# Autodesk Inventor assembly: chess-set-one
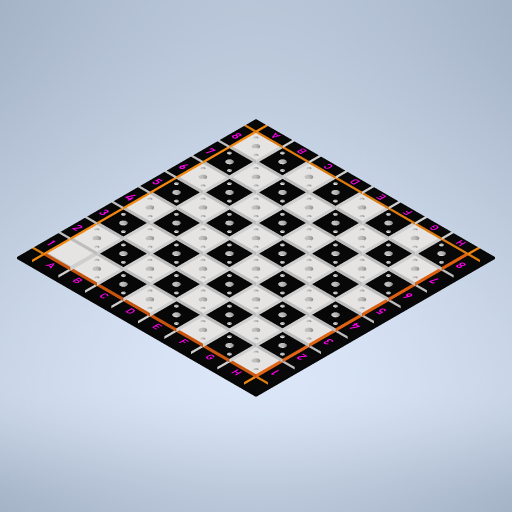
[picture p0: Inventor's stored thumbnail of the model, 512x512]
Saved by Autodesk Inventor 2024.1 (Build 281209000, 209)
## iProperties
Created: 2025-07-31
Part Number: chess-set-one
Document SubType Name: Assembly
Designer: iwheard
Author: iwheard
## Documents named in this file (8)
- C:\Users\iwheard\Documents\0004-CAD\3D-cad-main\chess-set\chess-set-one.iam
- C:\Users\iwheard\Documents\0004-CAD\3D-cad-main\chess-set\board.ipt
- C:\Users\iwheard\Documents\0004-CAD\3D-cad-main\chess-set\pawn-white-v2.ipt
- C:\Users\iwheard\Documents\0004-CAD\3D-cad-main\chess-set\queen-white.ipt
- C:\Users\iwheard\Documents\0004-CAD\3D-cad-main\chess-set\king-white.ipt
- C:\Users\iwheard\Documents\0004-CAD\3D-cad-main\chess-set\bishop-white.ipt
- C:\Users\iwheard\Documents\0004-CAD\3D-cad-main\chess-set\knight-white.ipt
- C:\Users\iwheard\Documents\0004-CAD\3D-cad-main\chess-set\rook-white.ipt
## Components (7 placed, 7 different names)
1. board:1 — Mate:1, Angle:1, Mate:2, Mate:3, Mate:4, Mate:5, Mate:6, Mate:7
2. pawn-white-v2:1 — Mate:1, Angle:1, Mate:7
3. queen-white:1 — Mate:3
4. king-white:1 — Mate:2
5. bishop-white:1 — Mate:4
6. knight-white:1 — Mate:5
7. rook-white:1 — Mate:6
## Relationships (8: Mate 7, Angle 1)
- Mate:1: board:1 ↔ pawn-white-v2:1
- Angle:1 (0 deg): board:1 ↔ pawn-white-v2:1
- Mate:2: board:1 ↔ king-white:1
- Mate:3: board:1 ↔ queen-white:1
- Mate:4: board:1 ↔ bishop-white:1
- Mate:5: board:1 ↔ knight-white:1
- Mate:6: board:1 ↔ rook-white:1
- Mate:7: board:1 ↔ pawn-white-v2:1
